# Autodesk Inventor assembly: MGN9H_250mm
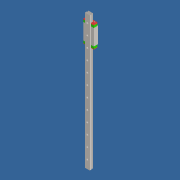
[picture p0: Inventor's stored thumbnail of the model, 180x180]
Saved by Autodesk Inventor 2020 (Build 240168000, 168)
## iProperties
Created: 2021-05-02
Part Number: MGN9H_250mm
Document SubType Name: Assembly
Designer: ken113
Author: ken113
## Documents named in this file (3)
- D:\Document\Github\Cheap_Belt_Printer\Model\Parts\Linear_Guide\MGN9H_250mm\MGN9H_250mm.iam
- D:\Document\Github\Cheap_Belt_Printer\Model\Parts\Linear_Guide\MGN9H_250mm\MGN9 LINEAR GUIDE RAIL, CONFIGURABLE, 250 mm.ipt
- D:\Document\Github\Cheap_Belt_Printer\Model\Parts\Linear_Guide\MGN9H_250mm\MGN9H, LINEAR GUIDE BLOCK.ipt
## Components (2 placed, 2 different names)
1. MGN9 LINEAR GUIDE RAIL, CONFIGURABLE, 250 mm:1 — メイト:1, メイト:2
2. MGN9H, LINEAR GUIDE BLOCK:1 — メイト:1, メイト:2
## Relationships (2: Mate 2)
- メイト:1 [Mate]: MGN9 LINEAR GUIDE RAIL, CONFIGURABLE, 250 mm:1 ↔ MGN9H, LINEAR GUIDE BLOCK:1
- メイト:2 [Mate]: MGN9 LINEAR GUIDE RAIL, CONFIGURABLE, 250 mm:1 ↔ MGN9H, LINEAR GUIDE BLOCK:1
